# Autodesk Inventor assembly: Kit Frame Wide Base b
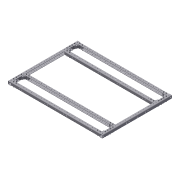
[picture p0: Inventor's stored thumbnail of the model, 180x180]
Saved by Autodesk Inventor 2013 (Build 170138000, 138)
## iProperties
Created: 2012-01-09
Part Number: Kit Frame Wide Base b
Document SubType Name: Assembly
Designer: Nemo
Author: Nemo
## Documents named in this file (5)
- \\lmss\students\Robotics\CAD Files\COTS Parts\Kit Frame - AndyMark\Kit Frame 28x38 Long.iam
- \\lmss\students\Robotics\CAD Files\COTS Parts\Kit Frame - AndyMark\C Channel.ipt
- \\lmss\students\Robotics\CAD Files\COTS Parts\Kit Frame - AndyMark\Components\C Channel Short for Long Base.ipt
- \\lmss\students\Robotics\CAD Files\COTS Parts\Kit Frame - AndyMark\Components\CornerConnectAssyLeft.iam
- \\lmss\students\Robotics\CAD Files\COTS Parts\Kit Frame - AndyMark\Components\CornerConnectAssyRight.iam
## Components (14 placed, 4 different names)
1. C Channel:1 — Flush:1, Flush:2, Mate:1, Mate:2, Flush:3, Flush:4, Mate:4, Flush:5, Mate:8, Flush:6, Flush:7, Insert:3, Mate:18, Insert:10
2. C Channel:2 — Mate:2, Flush:3, Insert:1, Mate:14, Mate:35
3. C Channel Short for Long Base:1 — Flush:4, Mate:4, Mate:15, Mate:32, Mate:33, Mate:34
4. C Channel Short for Long Base:2 — Flush:5, Mate:8, Mate:19, Mate:29, Mate:30, Insert:9, Insert:12
5. C Channel:3 — Flush:6, Insert:4, Mate:20, Mate:31
6. C Channel:4 — Flush:7, Insert:8, Mate:24, Insert:11
7. CornerConnectAssyLeft:1 [sub-assembly] — Insert:10, Mate:32
8. CornerConnectAssyRight:1 [sub-assembly] — Insert:1, Mate:14, Mate:15
9. CornerConnectAssyLeft:2 [sub-assembly] — Insert:9, Mate:31
10. CornerConnectAssyRight:2 [sub-assembly] — Insert:4, Mate:20, Mate:33
11. CornerConnectAssyLeft:3 [sub-assembly] — Insert:11, Mate:34
12. CornerConnectAssyRight:3 [sub-assembly] — Insert:3, Mate:18, Mate:19
13. CornerConnectAssyLeft:4 [sub-assembly] — Insert:12, Mate:35
14. CornerConnectAssyRight:4 [sub-assembly] — Insert:8, Mate:24, Mate:29, Mate:30
## Relationships (32: Mate 17, Insert 8, Flush 7)
- Flush:1 (-342.9 mm): C Channel:1
- Flush:2: C Channel:1
- Mate:1 (87.63 mm): C Channel:1
- Mate:2: C Channel:1 ↔ C Channel:2
- Flush:3: C Channel:1 ↔ C Channel:2
- Flush:4: C Channel:1 ↔ C Channel Short for Long Base:1
- Mate:4: C Channel:1 ↔ C Channel Short for Long Base:1
- Flush:5: C Channel:1 ↔ C Channel Short for Long Base:2
- Mate:8: C Channel:1 ↔ C Channel Short for Long Base:2
- Flush:6: C Channel:1 ↔ C Channel:3
- Flush:7: C Channel:1 ↔ C Channel:4
- Insert:1: C Channel:2 ↔ CornerConnectAssyRight:1
- Mate:14: C Channel:2 ↔ CornerConnectAssyRight:1
- Mate:15: C Channel Short for Long Base:1 ↔ CornerConnectAssyRight:1
- Insert:3: C Channel:1 ↔ CornerConnectAssyRight:3
- Mate:18: C Channel:1 ↔ CornerConnectAssyRight:3
- Mate:19: C Channel Short for Long Base:2 ↔ CornerConnectAssyRight:3
- Insert:4: C Channel:3 ↔ CornerConnectAssyRight:2
- Mate:20: C Channel:3 ↔ CornerConnectAssyRight:2
- Insert:8: C Channel:4 ↔ CornerConnectAssyRight:4
- Mate:24: C Channel:4 ↔ CornerConnectAssyRight:4
- Mate:29: C Channel Short for Long Base:2 ↔ CornerConnectAssyRight:4
- Mate:30: C Channel Short for Long Base:2 ↔ CornerConnectAssyRight:4
- Insert:9: C Channel Short for Long Base:2 ↔ CornerConnectAssyLeft:2
- Mate:31: C Channel:3 ↔ CornerConnectAssyLeft:2
- Insert:10: C Channel:1 ↔ CornerConnectAssyLeft:1
- Mate:32: C Channel Short for Long Base:1 ↔ CornerConnectAssyLeft:1
- Mate:33: C Channel Short for Long Base:1 ↔ CornerConnectAssyRight:2
- Insert:11: C Channel:4 ↔ CornerConnectAssyLeft:3
- Mate:34: C Channel Short for Long Base:1 ↔ CornerConnectAssyLeft:3
- Insert:12: C Channel Short for Long Base:2 ↔ CornerConnectAssyLeft:4
- Mate:35: C Channel:2 ↔ CornerConnectAssyLeft:4
